# Autodesk Inventor assembly: Shoulder_nema24_v2
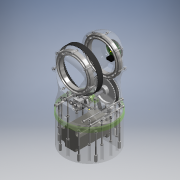
[picture p0: Inventor's stored thumbnail of the model, 180x180]
Saved by Autodesk Inventor 2016 (Build 200138000, 138)
## iProperties
Created: 2015-01-06
Part Number: Shoulder_nema24_v2
Document SubType Name: Assembly
Designer: 4ndreas
Mass: 6208.8 g
Surface Area: 5974.67 cm^2
Volume: 2503.18 cm^3
Density: 2.48036 g/cm^3
Author: 4ndreas
## Documents named in this file (30)
- C:\Users\4ndreas\Documents\Inventor\RobotARM v2\v4\Shoulder_nema24_v2.iam
- C:\Users\4ndreas\Documents\Inventor\RobotARM v2\v2\BaseJoint\Konstruktions-Assistent\Übertragung des Zahnriemens1.iam
- C:\Users\4ndreas\Documents\Inventor\Content Center Files\R2014\de-DE\DIN 125-1  A\DIN 125 - A 4,3.ipt
- C:\Users\4ndreas\Documents\Inventor\Content Center Files\R2014\de-DE\DIN BEARING(1)\DIN 625 SKF - SKF 624.ipt
- C:\Users\4ndreas\Documents\Inventor\Content Center Files\R2014\de-DE\DIN 934\DIN 934 - M4 x 0,7.ipt
- C:\Users\4ndreas\Documents\Inventor\RobotARM v2\v2\encoder.iam
- C:\Users\4ndreas\Documents\Inventor\Content Center Files\R2014\de-DE\DIN 912\DIN 912 - M4 x 0,7 x 35 x 20.ipt
- C:\Users\4ndreas\Documents\Inventor\RobotARM v2\v4\Shoulder_stepper\Konstruktions-Assistent\Übertragung des Zahnriemens1.iam
- C:\Users\4ndreas\Documents\Inventor\Content Center Files\R2014\de-DE\DIN BEARING(1)\DIN 625 SKF - SKF 61818.ipt
- C:\Users\4ndreas\Documents\Inventor\RobotARM v2\v4\Shoulder_basis_N24.ipt
- C:\Users\4ndreas\Documents\Inventor\RobotARM v2\v4\CoverBase.ipt
- C:\Users\4ndreas\Documents\Inventor\RobotARM v2\v4\Shoulder_nema24_v2\Konstruktions-Assistent\Welle1.iam
- C:\Users\4ndreas\Documents\Inventor\RobotARM v2\v4\Nema24_100.ipt
- C:\Users\4ndreas\Documents\Inventor\Content Center Files\R2014\de-DE\DIN BEARING(1)\DIN 625 SKF - SKF 608.ipt
- C:\Users\4ndreas\Documents\Inventor\Content Center Files\R2014\de-DE\DIN 125-1  A\DIN 125 - A 8,4.ipt
- C:\Users\4ndreas\Documents\Inventor\RobotARM v2\v4\LagerKlemme.ipt
- C:\Users\4ndreas\Documents\Inventor\RobotARM v2\v4\16221600.ipt
- C:\Users\4ndreas\Documents\Inventor\RobotARM v2\v4\Synchrone RiemenscheibeT5_z48.ipt
- C:\Users\4ndreas\Documents\Inventor\RobotARM v2\v4\Alu_Belt_tens.ipt
- C:\Users\4ndreas\Documents\Inventor\Content Center Files\R2014\de-DE\DIN 9021\DIN 9021 - 4,3.ipt
- C:\Users\4ndreas\Documents\Inventor\RobotARM v2\v4\DIN 912 - M4 x 0,7.ipt
- C:\Users\4ndreas\Documents\Inventor\Content Center Files\R2014\de-DE\DIN 912\DIN 912 - M4 x 0,7 x 20 x 18,25.ipt
- C:\Users\4ndreas\Documents\Inventor\Content Center Files\R2014\de-DE\DIN 912\DIN 912 - M4 x 0,7 x 25 x 23,25.ipt
- C:\Users\4ndreas\Documents\Inventor\RobotARM v2\v4\DIN 912 - M4 x 0,7 x 70.ipt
- C:\Users\4ndreas\Documents\Inventor\RobotARM v2\Diszanzbolzen_M4x20.ipt
- C:\Users\4ndreas\Documents\Inventor\Content Center Files\R2014\de-DE\DIN 562\DIN 562 - M4 x 7.ipt
- C:\Users\4ndreas\Documents\Inventor\Content Center Files\R2014\de-DE\DIN 912\DIN 912 - M4 x 0,7 x 30 x 20.ipt
- C:\Users\4ndreas\Documents\Inventor\RobotARM v2\v4\DIN 912 - M4 x 0,7 x 60.ipt
- C:\Users\4ndreas\Documents\Inventor\Content Center Files\R2014\de-DE\DIN 7991(2)\DIN 7991 - M3x25.ipt
- C:\Users\4ndreas\Documents\Inventor\Content Center Files\R2014\de-DE\DIN 934\DIN 934 - M3 x 0,5.ipt
## Components (141 placed, 28 different names)
1. Übertragung des Zahnriemens:1 [sub-assembly] — Passend:1, Passend:12, Passend:49, Passend:138, Fluchtend:18, Passend:147, Passend:173, Passend:195, Passend:228, Passend:229
2. DIN 912 - ersetzt durch DIN EN ISO 4762 M4 x 50:1 — Passend:69, Passend:82, Passend:99, Passend:179, Passend:198, Passend:203, Passend:209, Passend:210
3. DIN 625 SKF SKF 624:1 — Passend:178, Passend:192
4. DIN 625 SKF SKF 624:2 — Passend:177, Passend:186, Passend:188
5. DIN 625 SKF SKF 624:3 — Passend:80, Passend:82, Passend:181
6. DIN 625 SKF SKF 624:4 — Passend:80, Passend:180, Passend:212
7. DIN 125-1 A A 4,3:3 — Passend:193, Passend:219
8. DIN 125-1 A A 4,3:4 — Passend:183
9. DIN 125-1 A A 4,3:6 — Passend:189, Passend:194
10. DIN 934 - ersetzt durch DIN EN 24032/28673/28674 M4:1 — Passend:99, Passend:183
11. encoder:2 [sub-assembly] — Passend:116, Passend:162, Passend:163
12. Übertragung des Zahnriemens:2 [sub-assembly] — Passend:130, Passend:182
13. Nema24_100:1 — Passend:130, Winkel:10, Passend:174, Passend:175, Passend:255
14. DIN 625 SKF SKF 61818:1 — Passend:138, Passend:142, Tangential:2
15. Shoulder_basis_N24:1 — Passend:139, Fluchtend:14, Passend:140, Fluchtend:16, Passend:142, Passend:143, Passend:144, Fluchtend:17, Passend:162, Passend:163, Passend:164, Passend:169, Fluchtend:19, Passend:182, Passend:69, Passend:191, Fluchtend:20, Passend:204, Passend:205, Passend:206, Passend:208, Passend:213, Passend:221, Passend:224, Passend:225, Passend:226, Passend:227, Passend:230, Passend:293, Passend:294, Passend:295, Passend:296, Passend:297, Passend:298, Passend:299, Passend:300, Passend:301, Passend:302, Passend:303, Passend:304, Passend:305, Passend:306, Passend:307, Passend:308, Passend:309, Passend:310, Passend:311, Passend:328, Passend:329, Passend:330, Passend:331, Passend:332, Passend:333, Passend:334, Passend:335, Passend:336, Passend:337, Passend:338, Passend:339, Passend:340, Passend:341, Passend:342, Passend:344, Passend:345, Passend:346, Passend:353, Passend:354, Passend:355, Passend:356, Passend:357, Passend:358, Passend:359, Passend:367, Passend:369, Passend:370, Passend:371, Passend:374, Passend:375
16. CoverBase:1 — Passend:143, Passend:164, Passend:230, Passend:231, Passend:232, Passend:233, Passend:234, Passend:239, Passend:240, Passend:241, Passend:242, Passend:247, Passend:248, Passend:249, Passend:250, Passend:255, Passend:256, Passend:257, Passend:258, Passend:259, Passend:260, Passend:261, Passend:262, Passend:263, Passend:264, Passend:265, Passend:266, Passend:267, Passend:268, Passend:269, Passend:271, Passend:272, Passend:273, Passend:274, Passend:275, Passend:276, Passend:277, Passend:278, Passend:279, Passend:280, Passend:281, Passend:282, Passend:283, Passend:284, Passend:285, Fluchtend:31, Fluchtend:32, Passend:286, Fluchtend:33, Fluchtend:34, Fluchtend:35, Fluchtend:36, Fluchtend:37
17. DIN 625 SKF SKF 61818:2 — Passend:144, Fluchtend:17, Tangential:1
18. Welle:1 [sub-assembly] — Fluchtend:18, Passend:147, Passend:153, Passend:154, Passend:155, Passend:165, Passend:166
19. DIN 625 SKF SKF 608:1 — Passend:153, Passend:167, Passend:169
20. DIN 625 SKF SKF 608:3 — Passend:154, Passend:170, Passend:171
21. DIN 625 SKF SKF 608:4 — Passend:155
22. Synchrone RiemenscheibeT5_z48:1 — Passend:165, Passend:172
23. DIN 125-1 A A 8,4:1 — Passend:166, Passend:167, Passend:172
24. DIN 125-1 A A 8,4:2 — Passend:170, Passend:171, Passend:173
25. LagerKlemme:1 — Fluchtend:19, Passend:226, Passend:227, Passend:324, Passend:325, Passend:326, Passend:327
26. 16221600:1 — Passend:174, Passend:175
27. DIN 625 SKF SKF 624:5 — Passend:177, Passend:178, Passend:190
28. DIN 625 SKF SKF 624:6 — Passend:179, Passend:180, Passend:181
29. Alu_Belt_tens:1 — Passend:186, Passend:191, Passend:196, Passend:197, Fluchtend:20, Passend:222
30. DIN 912 - ersetzt durch DIN EN ISO 4762 M4 x 20:1 — Passend:197, Passend:200, Passend:201
31. DIN 912 - ersetzt durch DIN EN ISO 4762 M4 x 20:2 — Passend:196, Passend:199, Passend:202
32. DIN 912 - ersetzt durch DIN EN ISO 4762 M4 x 35:5 — Passend:188, Passend:189, Passend:190, Passend:192, Passend:193, Passend:194, Passend:195, Passend:207, Passend:218
33. DIN 9021 4,3:1 — Passend:198, Passend:203, Passend:204
34. DIN 9021 4,3:2 — Passend:200, Passend:201, Passend:205
35. DIN 9021 4,3:3 — Passend:199, Passend:202, Passend:206
36. DIN 9021 4,3:4 — Passend:207, Passend:208, Passend:220
37. DIN 9021 4,3:5 — Passend:209, Passend:211, Passend:213
38. DIN 934 - ersetzt durch DIN EN 24032/28673/28674 M4:2 — Passend:210, Passend:211, Passend:212
39. DIN 125-1 A A 4,3:7 — Passend:215, Passend:217, Passend:220
40. DIN 125-1 A A 4,3:8 — Passend:214, Passend:215, Passend:216
41. DIN 125-1 A A 4,3:9 — Passend:214, Passend:216, Passend:217, Passend:218, Passend:219
42. DIN 912 - ersetzt durch DIN EN ISO 4762 M4 x 25:1 — Passend:221, Passend:222, Passend:223
43. DIN 934 - ersetzt durch DIN EN 24032/28673/28674 M4:3 — Passend:223, Passend:224, Passend:225
44. DIN 912 - ersetzt durch DIN EN ISO 4762 M4 x 25:2 — Passend:233, Passend:235, Passend:245
45. DIN 912 - ersetzt durch DIN EN ISO 4762 M4 x 25:3 — Passend:232, Passend:237, Passend:243
46. DIN 912 - ersetzt durch DIN EN ISO 4762 M4 x 25:4 — Passend:231, Passend:236, Passend:244
47. DIN 912 - ersetzt durch DIN EN ISO 4762 M4 x 25:5 — Passend:234, Passend:238, Passend:246
48. DIN 125-1 A A 4,3:10 — Passend:238, Passend:239, Passend:246
49. DIN 125-1 A A 4,3:11 — Passend:237, Passend:241, Passend:243
50. DIN 125-1 A A 4,3:12 — Passend:235, Passend:242, Passend:245
51. DIN 125-1 A A 4,3:13 — Passend:236, Passend:240, Passend:244
52. DIN 625 SKF SKF 624:7 — Passend:248, Passend:251, Passend:252
53. DIN 625 SKF SKF 624:8 — Passend:247, Passend:251, Passend:253, Passend:254
54. DIN 125-1 A A 4,3:14 — Passend:249, Passend:250, Passend:252
55. DIN 125-1 A A 4,3:15 — Passend:253, Passend:254
56. DIN 912 - ersetzt durch DIN EN ISO 4762 M4 x 70:1 — Passend:259, Fluchtend:24, Fluchtend:25, Passend:291
57. DIN 912 - ersetzt durch DIN EN ISO 4762 M4 x 70:2 — Passend:263, Fluchtend:29, Passend:314
58. DIN 912 - ersetzt durch DIN EN ISO 4762 M4 x 70:3 — Passend:262, Fluchtend:29, Fluchtend:30, Passend:313
59. DIN 912 - ersetzt durch DIN EN ISO 4762 M4 x 70:4 — Passend:261, Fluchtend:28, Fluchtend:30, Passend:312
60. DIN 912 - ersetzt durch DIN EN ISO 4762 M4 x 70:5 — Passend:260, Fluchtend:25, Passend:292
61. DIN 912 - ersetzt durch DIN EN ISO 4762 M4 x 70:6 — Passend:258, Fluchtend:26, Fluchtend:27, Passend:316
62. DIN 912 - ersetzt durch DIN EN ISO 4762 M4 x 70:7 — Passend:257, Fluchtend:27, Fluchtend:28, Passend:317
63. DIN 912 - ersetzt durch DIN EN ISO 4762 M4 x 70:8 — Passend:256, Fluchtend:23, Fluchtend:24, Passend:290
64. DIN 912 - ersetzt durch DIN EN ISO 4762 M4 x 70:11 — Passend:267, Fluchtend:21, Passend:287
65. DIN 912 - ersetzt durch DIN EN ISO 4762 M4 x 70:12 — Passend:266, Fluchtend:21, Fluchtend:22, Passend:288
66. DIN 912 - ersetzt durch DIN EN ISO 4762 M4 x 70:13 — Passend:265, Fluchtend:22, Fluchtend:23, Passend:289
67. DIN 912 - ersetzt durch DIN EN ISO 4762 M4 x 70:14 — Passend:264, Fluchtend:26, Passend:315
68. DIN 912 - ersetzt durch DIN EN ISO 4762 M4 x 70:15 — Passend:268, Passend:269, Passend:270, Fluchtend:45, Fluchtend:46
69. Diszanzbolzen_M4x20:1 — Passend:270, Passend:278, Passend:279
70. Diszanzbolzen_M4x20:2 — Passend:271, Passend:283, Fluchtend:36, Passend:366
71. Diszanzbolzen_M4x20:3 — Passend:272, Passend:284, Fluchtend:37, Passend:365
72. Diszanzbolzen_M4x20:4 — Passend:276, Passend:281, Fluchtend:34, Passend:361
73. Diszanzbolzen_M4x20:5 — Passend:275, Passend:280, Fluchtend:33, Passend:362
74. Diszanzbolzen_M4x20:6 — Passend:274, Fluchtend:32, Passend:286, Passend:363
75. Diszanzbolzen_M4x20:7 — Passend:273, Passend:285, Fluchtend:31, Passend:364
76. Diszanzbolzen_M4x20:8 — Passend:277, Passend:282, Fluchtend:35, Passend:360
77. DIN 934 - ersetzt durch DIN EN 24032/28673/28674 M4:4 — Passend:287, Fluchtend:42, Passend:293
78. DIN 934 - ersetzt durch DIN EN 24032/28673/28674 M4:5 — Passend:288, Fluchtend:40, Fluchtend:41, Passend:294
79. DIN 934 - ersetzt durch DIN EN 24032/28673/28674 M4:6 — Passend:289, Fluchtend:41, Fluchtend:42, Passend:295
80. DIN 934 - ersetzt durch DIN EN 24032/28673/28674 M4:7 — Passend:290, Fluchtend:38, Passend:296
81. DIN 934 - ersetzt durch DIN EN 24032/28673/28674 M4:10 — Passend:292, Fluchtend:39, Fluchtend:40, Passend:298
82. DIN 934 - ersetzt durch DIN EN 24032/28673/28674 M4:11 — Passend:291, Fluchtend:38, Fluchtend:39, Passend:297, Passend:299
83. DIN 562 M4:1 — Passend:300, Passend:301, Passend:317
84. DIN 562 M4:2 — Passend:302, Passend:303, Passend:316
85. DIN 562 M4:3 — Passend:304, Passend:305, Passend:315
86. DIN 562 M4:4 — Passend:307, Passend:310, Passend:313
87. DIN 562 M4:5 — Passend:306, Passend:311, Passend:312
88. DIN 562 M4:6 — Passend:308, Passend:309, Passend:314
89. DIN 912 - ersetzt durch DIN EN ISO 4762 M4 x 30:1 — Passend:318, Passend:321, Passend:322, Passend:324
90. DIN 912 - ersetzt durch DIN EN ISO 4762 M4 x 30:2 — Passend:319, Passend:320, Passend:323, Passend:326
91. DIN 934 - ersetzt durch DIN EN 24032/28673/28674 M4:12 — Passend:319, Fluchtend:43, Passend:329
92. DIN 934 - ersetzt durch DIN EN 24032/28673/28674 M4:13 — Passend:318, Fluchtend:43, Passend:328, Passend:330
93. DIN 125-1 A A 4,3:16 — Passend:321, Passend:322, Passend:325
94. DIN 125-1 A A 4,3:17 — Passend:320, Passend:323, Passend:327
95. Diszanzbolzen_M4x20:9 — Passend:333, Passend:339, Passend:342, Passend:347
96. Diszanzbolzen_M4x20:10 — Passend:334, Passend:340, Passend:341, Passend:351
97. Diszanzbolzen_M4x20:11 — Passend:331, Passend:335, Passend:338, Passend:349
98. Diszanzbolzen_M4x20:12 — Passend:332, Passend:336, Passend:337
99. DIN 912 - ersetzt durch DIN EN ISO 4762 M4 x 50:2 — Passend:344, Passend:346
100. DIN 912 - ersetzt durch DIN EN ISO 4762 M4 x 50:3 — Passend:347, Passend:348, Passend:359
101. DIN 912 - ersetzt durch DIN EN ISO 4762 M4 x 50:4 — Passend:348, Passend:353
102. DIN 912 - ersetzt durch DIN EN ISO 4762 M4 x 50:5 — Passend:345, Passend:356
103. DIN 912 - ersetzt durch DIN EN ISO 4762 M4 x 60:16 — Passend:350, Passend:355
104. DIN 912 - ersetzt durch DIN EN ISO 4762 M4 x 60:17 — Passend:349, Passend:350, Passend:357
105. DIN 912 - ersetzt durch DIN EN ISO 4762 M4 x 60:18 — Passend:352, Passend:354
106. DIN 912 - ersetzt durch DIN EN ISO 4762 M4 x 60:19 — Passend:351, Passend:352, Passend:358
107. DIN 912 - ersetzt durch DIN EN ISO 4762 M4 x 70:20 — Passend:361, Fluchtend:47, Fluchtend:48, Fluchtend:49
108. DIN 912 - ersetzt durch DIN EN ISO 4762 M4 x 70:21 — Passend:362, Fluchtend:47
109. DIN 912 - ersetzt durch DIN EN ISO 4762 M4 x 70:22 — Passend:364, Fluchtend:50
110. DIN 912 - ersetzt durch DIN EN ISO 4762 M4 x 70:24 — Passend:363, Fluchtend:49, Fluchtend:50
111. DIN 912 - ersetzt durch DIN EN ISO 4762 M4 x 70:25 — Passend:360, Fluchtend:46, Fluchtend:48
112. DIN 912 - ersetzt durch DIN EN ISO 4762 M4 x 70:26 — Passend:365, Fluchtend:44
113. DIN 912 - ersetzt durch DIN EN ISO 4762 M4 x 70:27 — Passend:366, Fluchtend:44, Fluchtend:45
114. DIN 934 - ersetzt durch DIN EN 24032/28673/28674 M3:1 — Passend:368, Passend:369, Passend:370
115. DIN 7991 M3x25:1 — Passend:367, Tangential:1, Passend:368
116. DIN 934 - ersetzt durch DIN EN 24032/28673/28674 M3:2
117. DIN 7991 M3x25:2
118. DIN 934 - ersetzt durch DIN EN 24032/28673/28674 M3:3
119. DIN 7991 M3x25:3
120. DIN 934 - ersetzt durch DIN EN 24032/28673/28674 M3:4
121. DIN 7991 M3x25:4
122. DIN 934 - ersetzt durch DIN EN 24032/28673/28674 M3:5
123. DIN 7991 M3x25:5
124. DIN 934 - ersetzt durch DIN EN 24032/28673/28674 M3:6
125. DIN 7991 M3x25:6
126. DIN 934 - ersetzt durch DIN EN 24032/28673/28674 M3:7
127. DIN 7991 M3x25:7
128. DIN 7991 M3x25:8 — Passend:371, Passend:373, Tangential:2
129. DIN 934 - ersetzt durch DIN EN 24032/28673/28674 M3:8 — Passend:373, Passend:374, Passend:375
130. DIN 7991 M3x25:9
131. DIN 934 - ersetzt durch DIN EN 24032/28673/28674 M3:9
132. DIN 7991 M3x25:10
133. DIN 934 - ersetzt durch DIN EN 24032/28673/28674 M3:10
134. DIN 7991 M3x25:11
135. DIN 934 - ersetzt durch DIN EN 24032/28673/28674 M3:11
136. DIN 7991 M3x25:12
137. DIN 934 - ersetzt durch DIN EN 24032/28673/28674 M3:12
138. DIN 7991 M3x25:13
139. DIN 934 - ersetzt durch DIN EN 24032/28673/28674 M3:13
140. DIN 7991 M3x25:14
141. DIN 934 - ersetzt durch DIN EN 24032/28673/28674 M3:14
## Component patterns: (7 elements, first: DIN 934 - ersetzt durch DIN EN 24032/28673/28674 M3:1 + DIN 7991 M3x25:1), (7 elements, first: DIN 7991 M3x25:8 + DIN 934 - ersetzt durch DIN EN 24032/28673/28674 M3:8)
## Relationships (274: Mate 233, Flush 38, Tangent 2, Angle 1)
- Passend:1 [Mate]: Übertragung des Zahnriemens:1
- Passend:4 [Mate]
- Passend:12 [Mate]: Übertragung des Zahnriemens:1
- Passend:49 [Mate]: Übertragung des Zahnriemens:1
- Passend:62 [Mate]
- Passend:63 [Mate]
- Passend:69 [Mate]: DIN 912 - ersetzt durch DIN EN ISO 4762 M4 x 50:1 ↔ Shoulder_basis_N24:1
- Passend:80 [Mate]: DIN 625 SKF SKF 624:3 ↔ DIN 625 SKF SKF 624:4
- Passend:82 [Mate]: DIN 912 - ersetzt durch DIN EN ISO 4762 M4 x 50:1 ↔ DIN 625 SKF SKF 624:3
- [Mate]: DIN 912 - ersetzt durch DIN EN ISO 4762 M4 x 50:1 ↔ DIN 125-1 A A 4,3:4
- [Mate]: DIN 625 SKF SKF 624:3 ↔ DIN 125-1 A A 4,3:4
- [Mate]: DIN 625 SKF SKF 624:2 ↔ DIN 125-1 A A 4,3:6
- [Mate]: DIN 625 SKF SKF 624:1 ↔ DIN 125-1 A A 4,3:3
- Passend:99 [Mate]: DIN 912 - ersetzt durch DIN EN ISO 4762 M4 x 50:1 ↔ DIN 934 - ersetzt durch DIN EN 24032/28673/28674 M4:1
- Passend:116 [Mate]: encoder:2
- Fluchtend:12 [Flush] (43 mm)
- Fluchtend:13 [Flush] (20 mm)
- Passend:130 [Mate]: Übertragung des Zahnriemens:2 ↔ Nema24_100:1
- Winkel:10 [Angle] (0 deg): Nema24_100:1
- Passend:138 [Mate]: Übertragung des Zahnriemens:1 ↔ DIN 625 SKF SKF 61818:1
- Passend:139 [Mate]: Shoulder_basis_N24:1
- Fluchtend:14 [Flush]: Shoulder_basis_N24:1
- Passend:140 [Mate]: Shoulder_basis_N24:1
- Fluchtend:16 [Flush]: Shoulder_basis_N24:1
- Passend:142 [Mate]: DIN 625 SKF SKF 61818:1 ↔ Shoulder_basis_N24:1
- Passend:143 [Mate]: Shoulder_basis_N24:1 ↔ CoverBase:1
- Passend:144 [Mate]: Shoulder_basis_N24:1 ↔ DIN 625 SKF SKF 61818:2
- Fluchtend:17 [Flush]: Shoulder_basis_N24:1 ↔ DIN 625 SKF SKF 61818:2
- Fluchtend:18 [Flush] (-10 mm): Übertragung des Zahnriemens:1 ↔ Welle:1
- Passend:147 [Mate]: Übertragung des Zahnriemens:1 ↔ Welle:1
- Passend:153 [Mate]: Welle:1 ↔ DIN 625 SKF SKF 608:1
- Passend:154 [Mate]: Welle:1 ↔ DIN 625 SKF SKF 608:3
- Passend:155 [Mate]: Welle:1 ↔ DIN 625 SKF SKF 608:4
- Passend:162 [Mate]: encoder:2 ↔ Shoulder_basis_N24:1
- Passend:163 [Mate]: encoder:2 ↔ Shoulder_basis_N24:1
- Passend:164 [Mate]: Shoulder_basis_N24:1 ↔ CoverBase:1
- Passend:165 [Mate]: Welle:1 ↔ Synchrone RiemenscheibeT5_z48:1
- Passend:166 [Mate]: Welle:1 ↔ DIN 125-1 A A 8,4:1
- Passend:167 [Mate]: DIN 625 SKF SKF 608:1 ↔ DIN 125-1 A A 8,4:1
- Passend:169 [Mate]: Shoulder_basis_N24:1 ↔ DIN 625 SKF SKF 608:1
- Passend:170 [Mate]: DIN 625 SKF SKF 608:3 ↔ DIN 125-1 A A 8,4:2
- Passend:171 [Mate]: DIN 625 SKF SKF 608:3 ↔ DIN 125-1 A A 8,4:2
- Passend:172 [Mate]: Synchrone RiemenscheibeT5_z48:1 ↔ DIN 125-1 A A 8,4:1
- Passend:173 [Mate] (0.5 mm): Übertragung des Zahnriemens:1 ↔ DIN 125-1 A A 8,4:2
- Fluchtend:19 [Flush]: Shoulder_basis_N24:1 ↔ LagerKlemme:1
- Passend:174 [Mate]: Nema24_100:1 ↔ 16221600:1
- Passend:175 [Mate] (0.5 mm): Nema24_100:1 ↔ 16221600:1
- Passend:177 [Mate]: DIN 625 SKF SKF 624:2 ↔ DIN 625 SKF SKF 624:5
- Passend:178 [Mate]: DIN 625 SKF SKF 624:1 ↔ DIN 625 SKF SKF 624:5
- Passend:179 [Mate]: DIN 912 - ersetzt durch DIN EN ISO 4762 M4 x 50:1 ↔ DIN 625 SKF SKF 624:6
- Passend:180 [Mate]: DIN 625 SKF SKF 624:4 ↔ DIN 625 SKF SKF 624:6
- Passend:181 [Mate]: DIN 625 SKF SKF 624:3 ↔ DIN 625 SKF SKF 624:6
- Passend:182 [Mate]: Übertragung des Zahnriemens:2 ↔ Shoulder_basis_N24:1
- Passend:183 [Mate]: DIN 125-1 A A 4,3:4 ↔ DIN 934 - ersetzt durch DIN EN 24032/28673/28674 M4:1
- Passend:186 [Mate]: DIN 625 SKF SKF 624:2 ↔ Alu_Belt_tens:1
- Passend:188 [Mate]: DIN 625 SKF SKF 624:2 ↔ DIN 912 - ersetzt durch DIN EN ISO 4762 M4 x 35:5
- Passend:189 [Mate]: DIN 125-1 A A 4,3:6 ↔ DIN 912 - ersetzt durch DIN EN ISO 4762 M4 x 35:5
- Passend:190 [Mate]: DIN 625 SKF SKF 624:5 ↔ DIN 912 - ersetzt durch DIN EN ISO 4762 M4 x 35:5
- Passend:191 [Mate]: Shoulder_basis_N24:1 ↔ Alu_Belt_tens:1
- Passend:192 [Mate]: DIN 625 SKF SKF 624:1 ↔ DIN 912 - ersetzt durch DIN EN ISO 4762 M4 x 35:5
- Passend:193 [Mate]: DIN 125-1 A A 4,3:3 ↔ DIN 912 - ersetzt durch DIN EN ISO 4762 M4 x 35:5
- Passend:194 [Mate]: DIN 125-1 A A 4,3:6 ↔ DIN 912 - ersetzt durch DIN EN ISO 4762 M4 x 35:5
- Passend:195 [Mate]: Übertragung des Zahnriemens:1 ↔ DIN 912 - ersetzt durch DIN EN ISO 4762 M4 x 35:5
- Passend:196 [Mate]: Alu_Belt_tens:1 ↔ DIN 912 - ersetzt durch DIN EN ISO 4762 M4 x 20:2
- Passend:197 [Mate]: Alu_Belt_tens:1 ↔ DIN 912 - ersetzt durch DIN EN ISO 4762 M4 x 20:1
- Fluchtend:20 [Flush]: Shoulder_basis_N24:1 ↔ Alu_Belt_tens:1
- Passend:198 [Mate]: DIN 912 - ersetzt durch DIN EN ISO 4762 M4 x 50:1 ↔ DIN 9021 4,3:1
- Passend:199 [Mate]: DIN 912 - ersetzt durch DIN EN ISO 4762 M4 x 20:2 ↔ DIN 9021 4,3:3
- Passend:200 [Mate]: DIN 912 - ersetzt durch DIN EN ISO 4762 M4 x 20:1 ↔ DIN 9021 4,3:2
- Passend:201 [Mate]: DIN 912 - ersetzt durch DIN EN ISO 4762 M4 x 20:1 ↔ DIN 9021 4,3:2
- Passend:202 [Mate]: DIN 912 - ersetzt durch DIN EN ISO 4762 M4 x 20:2 ↔ DIN 9021 4,3:3
- Passend:203 [Mate]: DIN 912 - ersetzt durch DIN EN ISO 4762 M4 x 50:1 ↔ DIN 9021 4,3:1
- Passend:204 [Mate]: Shoulder_basis_N24:1 ↔ DIN 9021 4,3:1
- Passend:205 [Mate]: Shoulder_basis_N24:1 ↔ DIN 9021 4,3:2
- Passend:206 [Mate]: Shoulder_basis_N24:1 ↔ DIN 9021 4,3:3
- Passend:207 [Mate]: DIN 912 - ersetzt durch DIN EN ISO 4762 M4 x 35:5 ↔ DIN 9021 4,3:4
- Passend:208 [Mate]: Shoulder_basis_N24:1 ↔ DIN 9021 4,3:4
- Passend:209 [Mate]: DIN 912 - ersetzt durch DIN EN ISO 4762 M4 x 50:1 ↔ DIN 9021 4,3:5
- Passend:210 [Mate]: DIN 912 - ersetzt durch DIN EN ISO 4762 M4 x 50:1 ↔ DIN 934 - ersetzt durch DIN EN 24032/28673/28674 M4:2
- Passend:211 [Mate]: DIN 9021 4,3:5 ↔ DIN 934 - ersetzt durch DIN EN 24032/28673/28674 M4:2
- Passend:212 [Mate]: DIN 625 SKF SKF 624:4 ↔ DIN 934 - ersetzt durch DIN EN 24032/28673/28674 M4:2
- Passend:213 [Mate]: Shoulder_basis_N24:1 ↔ DIN 9021 4,3:5
- Passend:214 [Mate]: DIN 125-1 A A 4,3:8 ↔ DIN 125-1 A A 4,3:9
- Passend:215 [Mate]: DIN 125-1 A A 4,3:7 ↔ DIN 125-1 A A 4,3:8
- Passend:216 [Mate]: DIN 125-1 A A 4,3:8 ↔ DIN 125-1 A A 4,3:9
- Passend:217 [Mate]: DIN 125-1 A A 4,3:7 ↔ DIN 125-1 A A 4,3:9
- Passend:218 [Mate]: DIN 912 - ersetzt durch DIN EN ISO 4762 M4 x 35:5 ↔ DIN 125-1 A A 4,3:9
- Passend:219 [Mate]: DIN 125-1 A A 4,3:3 ↔ DIN 125-1 A A 4,3:9
- Passend:220 [Mate]: DIN 9021 4,3:4 ↔ DIN 125-1 A A 4,3:7
- Passend:221 [Mate]: Shoulder_basis_N24:1 ↔ DIN 912 - ersetzt durch DIN EN ISO 4762 M4 x 25:1
- Passend:222 [Mate]: Alu_Belt_tens:1 ↔ DIN 912 - ersetzt durch DIN EN ISO 4762 M4 x 25:1
- Passend:223 [Mate]: DIN 912 - ersetzt durch DIN EN ISO 4762 M4 x 25:1 ↔ DIN 934 - ersetzt durch DIN EN 24032/28673/28674 M4:3
- Passend:224 [Mate]: Shoulder_basis_N24:1 ↔ DIN 934 - ersetzt durch DIN EN 24032/28673/28674 M4:3
- Passend:225 [Mate]: Shoulder_basis_N24:1 ↔ DIN 934 - ersetzt durch DIN EN 24032/28673/28674 M4:3
- Passend:226 [Mate]: Shoulder_basis_N24:1 ↔ LagerKlemme:1
- Passend:227 [Mate]: Shoulder_basis_N24:1 ↔ LagerKlemme:1
- Passend:228 [Mate]: Übertragung des Zahnriemens:1
- Passend:229 [Mate]: Übertragung des Zahnriemens:1
- Passend:230 [Mate]: Shoulder_basis_N24:1 ↔ CoverBase:1
- Passend:231 [Mate]: CoverBase:1 ↔ DIN 912 - ersetzt durch DIN EN ISO 4762 M4 x 25:4
- Passend:232 [Mate]: CoverBase:1 ↔ DIN 912 - ersetzt durch DIN EN ISO 4762 M4 x 25:3
- Passend:233 [Mate]: CoverBase:1 ↔ DIN 912 - ersetzt durch DIN EN ISO 4762 M4 x 25:2
- Passend:234 [Mate]: CoverBase:1 ↔ DIN 912 - ersetzt durch DIN EN ISO 4762 M4 x 25:5
- Passend:235 [Mate]: DIN 912 - ersetzt durch DIN EN ISO 4762 M4 x 25:2 ↔ DIN 125-1 A A 4,3:12
- Passend:236 [Mate]: DIN 912 - ersetzt durch DIN EN ISO 4762 M4 x 25:4 ↔ DIN 125-1 A A 4,3:13
- Passend:237 [Mate]: DIN 912 - ersetzt durch DIN EN ISO 4762 M4 x 25:3 ↔ DIN 125-1 A A 4,3:11
- Passend:238 [Mate]: DIN 912 - ersetzt durch DIN EN ISO 4762 M4 x 25:5 ↔ DIN 125-1 A A 4,3:10
- Passend:239 [Mate]: CoverBase:1 ↔ DIN 125-1 A A 4,3:10
- Passend:240 [Mate]: CoverBase:1 ↔ DIN 125-1 A A 4,3:13
- Passend:241 [Mate]: CoverBase:1 ↔ DIN 125-1 A A 4,3:11
- Passend:242 [Mate]: CoverBase:1 ↔ DIN 125-1 A A 4,3:12
- Passend:243 [Mate]: DIN 912 - ersetzt durch DIN EN ISO 4762 M4 x 25:3 ↔ DIN 125-1 A A 4,3:11
- Passend:244 [Mate]: DIN 912 - ersetzt durch DIN EN ISO 4762 M4 x 25:4 ↔ DIN 125-1 A A 4,3:13
- Passend:245 [Mate]: DIN 912 - ersetzt durch DIN EN ISO 4762 M4 x 25:2 ↔ DIN 125-1 A A 4,3:12
- Passend:246 [Mate]: DIN 912 - ersetzt durch DIN EN ISO 4762 M4 x 25:5 ↔ DIN 125-1 A A 4,3:10
- Passend:247 [Mate]: CoverBase:1 ↔ DIN 625 SKF SKF 624:8
- Passend:248 [Mate]: CoverBase:1 ↔ DIN 625 SKF SKF 624:7
- Passend:249 [Mate]: CoverBase:1 ↔ DIN 125-1 A A 4,3:14
- Passend:250 [Mate]: CoverBase:1 ↔ DIN 125-1 A A 4,3:14
- Passend:251 [Mate]: DIN 625 SKF SKF 624:7 ↔ DIN 625 SKF SKF 624:8
- Passend:252 [Mate]: DIN 625 SKF SKF 624:7 ↔ DIN 125-1 A A 4,3:14
- Passend:253 [Mate]: DIN 625 SKF SKF 624:8 ↔ DIN 125-1 A A 4,3:15
- Passend:254 [Mate]: DIN 625 SKF SKF 624:8 ↔ DIN 125-1 A A 4,3:15
- Passend:255 [Mate]: Nema24_100:1 ↔ CoverBase:1
- Passend:256 [Mate]: CoverBase:1 ↔ DIN 912 - ersetzt durch DIN EN ISO 4762 M4 x 70:8
- Passend:257 [Mate]: CoverBase:1 ↔ DIN 912 - ersetzt durch DIN EN ISO 4762 M4 x 70:7
- Passend:258 [Mate]: CoverBase:1 ↔ DIN 912 - ersetzt durch DIN EN ISO 4762 M4 x 70:6
- Passend:259 [Mate]: CoverBase:1 ↔ DIN 912 - ersetzt durch DIN EN ISO 4762 M4 x 70:1
- Passend:260 [Mate]: CoverBase:1 ↔ DIN 912 - ersetzt durch DIN EN ISO 4762 M4 x 70:5
- Passend:261 [Mate]: CoverBase:1 ↔ DIN 912 - ersetzt durch DIN EN ISO 4762 M4 x 70:4
- Passend:262 [Mate]: CoverBase:1 ↔ DIN 912 - ersetzt durch DIN EN ISO 4762 M4 x 70:3
- Passend:263 [Mate]: CoverBase:1 ↔ DIN 912 - ersetzt durch DIN EN ISO 4762 M4 x 70:2
- Passend:264 [Mate]: CoverBase:1 ↔ DIN 912 - ersetzt durch DIN EN ISO 4762 M4 x 70:14
- Passend:265 [Mate]: CoverBase:1 ↔ DIN 912 - ersetzt durch DIN EN ISO 4762 M4 x 70:13
- Passend:266 [Mate]: CoverBase:1 ↔ DIN 912 - ersetzt durch DIN EN ISO 4762 M4 x 70:12
- Passend:267 [Mate]: CoverBase:1 ↔ DIN 912 - ersetzt durch DIN EN ISO 4762 M4 x 70:11
- Fluchtend:21 [Flush]: DIN 912 - ersetzt durch DIN EN ISO 4762 M4 x 70:11 ↔ DIN 912 - ersetzt durch DIN EN ISO 4762 M4 x 70:12
- Fluchtend:22 [Flush]: DIN 912 - ersetzt durch DIN EN ISO 4762 M4 x 70:12 ↔ DIN 912 - ersetzt durch DIN EN ISO 4762 M4 x 70:13
- Fluchtend:23 [Flush]: DIN 912 - ersetzt durch DIN EN ISO 4762 M4 x 70:8 ↔ DIN 912 - ersetzt durch DIN EN ISO 4762 M4 x 70:13
- Fluchtend:24 [Flush]: DIN 912 - ersetzt durch DIN EN ISO 4762 M4 x 70:1 ↔ DIN 912 - ersetzt durch DIN EN ISO 4762 M4 x 70:8
- Fluchtend:25 [Flush]: DIN 912 - ersetzt durch DIN EN ISO 4762 M4 x 70:1 ↔ DIN 912 - ersetzt durch DIN EN ISO 4762 M4 x 70:5
- Fluchtend:26 [Flush]: DIN 912 - ersetzt durch DIN EN ISO 4762 M4 x 70:6 ↔ DIN 912 - ersetzt durch DIN EN ISO 4762 M4 x 70:14
- Fluchtend:27 [Flush]: DIN 912 - ersetzt durch DIN EN ISO 4762 M4 x 70:6 ↔ DIN 912 - ersetzt durch DIN EN ISO 4762 M4 x 70:7
- Fluchtend:28 [Flush]: DIN 912 - ersetzt durch DIN EN ISO 4762 M4 x 70:4 ↔ DIN 912 - ersetzt durch DIN EN ISO 4762 M4 x 70:7
- Fluchtend:29 [Flush]: DIN 912 - ersetzt durch DIN EN ISO 4762 M4 x 70:2 ↔ DIN 912 - ersetzt durch DIN EN ISO 4762 M4 x 70:3
- Fluchtend:30 [Flush]: DIN 912 - ersetzt durch DIN EN ISO 4762 M4 x 70:3 ↔ DIN 912 - ersetzt durch DIN EN ISO 4762 M4 x 70:4
- Passend:268 [Mate]: CoverBase:1 ↔ DIN 912 - ersetzt durch DIN EN ISO 4762 M4 x 70:15
- Passend:269 [Mate]: CoverBase:1 ↔ DIN 912 - ersetzt durch DIN EN ISO 4762 M4 x 70:15
- Passend:270 [Mate]: DIN 912 - ersetzt durch DIN EN ISO 4762 M4 x 70:15 ↔ Diszanzbolzen_M4x20:1
- Passend:271 [Mate]: CoverBase:1 ↔ Diszanzbolzen_M4x20:2
- Passend:272 [Mate]: CoverBase:1 ↔ Diszanzbolzen_M4x20:3
- Passend:273 [Mate]: CoverBase:1 ↔ Diszanzbolzen_M4x20:7
- Passend:274 [Mate]: CoverBase:1 ↔ Diszanzbolzen_M4x20:6
- Passend:275 [Mate]: CoverBase:1 ↔ Diszanzbolzen_M4x20:5
- Passend:276 [Mate]: CoverBase:1 ↔ Diszanzbolzen_M4x20:4
- Passend:277 [Mate]: CoverBase:1 ↔ Diszanzbolzen_M4x20:8
- Passend:278 [Mate]: CoverBase:1 ↔ Diszanzbolzen_M4x20:1
- Passend:279 [Mate]: CoverBase:1 ↔ Diszanzbolzen_M4x20:1
- Passend:280 [Mate]: CoverBase:1 ↔ Diszanzbolzen_M4x20:5
- Passend:281 [Mate]: CoverBase:1 ↔ Diszanzbolzen_M4x20:4
- Passend:282 [Mate]: CoverBase:1 ↔ Diszanzbolzen_M4x20:8
- Passend:283 [Mate]: CoverBase:1 ↔ Diszanzbolzen_M4x20:2
- Passend:284 [Mate]: CoverBase:1 ↔ Diszanzbolzen_M4x20:3
- Passend:285 [Mate]: CoverBase:1 ↔ Diszanzbolzen_M4x20:7
- Fluchtend:31 [Flush]: CoverBase:1 ↔ Diszanzbolzen_M4x20:7
- Fluchtend:32 [Flush]: CoverBase:1 ↔ Diszanzbolzen_M4x20:6
- Passend:286 [Mate]: CoverBase:1 ↔ Diszanzbolzen_M4x20:6
- Fluchtend:33 [Flush]: CoverBase:1 ↔ Diszanzbolzen_M4x20:5
- Fluchtend:34 [Flush]: CoverBase:1 ↔ Diszanzbolzen_M4x20:4
- Fluchtend:35 [Flush]: CoverBase:1 ↔ Diszanzbolzen_M4x20:8
- Fluchtend:36 [Flush]: CoverBase:1 ↔ Diszanzbolzen_M4x20:2
- Fluchtend:37 [Flush]: CoverBase:1 ↔ Diszanzbolzen_M4x20:3
- Passend:287 [Mate]: DIN 912 - ersetzt durch DIN EN ISO 4762 M4 x 70:11 ↔ DIN 934 - ersetzt durch DIN EN 24032/28673/28674 M4:4
- Passend:288 [Mate]: DIN 912 - ersetzt durch DIN EN ISO 4762 M4 x 70:12 ↔ DIN 934 - ersetzt durch DIN EN 24032/28673/28674 M4:5
- Passend:289 [Mate]: DIN 912 - ersetzt durch DIN EN ISO 4762 M4 x 70:13 ↔ DIN 934 - ersetzt durch DIN EN 24032/28673/28674 M4:6
- Passend:290 [Mate]: DIN 912 - ersetzt durch DIN EN ISO 4762 M4 x 70:8 ↔ DIN 934 - ersetzt durch DIN EN 24032/28673/28674 M4:7
- Passend:291 [Mate]: DIN 912 - ersetzt durch DIN EN ISO 4762 M4 x 70:1 ↔ DIN 934 - ersetzt durch DIN EN 24032/28673/28674 M4:11
- Passend:292 [Mate]: DIN 912 - ersetzt durch DIN EN ISO 4762 M4 x 70:5 ↔ DIN 934 - ersetzt durch DIN EN 24032/28673/28674 M4:10
- Fluchtend:38 [Flush]: DIN 934 - ersetzt durch DIN EN 24032/28673/28674 M4:7 ↔ DIN 934 - ersetzt durch DIN EN 24032/28673/28674 M4:11
- Fluchtend:39 [Flush]: DIN 934 - ersetzt durch DIN EN 24032/28673/28674 M4:10 ↔ DIN 934 - ersetzt durch DIN EN 24032/28673/28674 M4:11
- Fluchtend:40 [Flush]: DIN 934 - ersetzt durch DIN EN 24032/28673/28674 M4:5 ↔ DIN 934 - ersetzt durch DIN EN 24032/28673/28674 M4:10
- Fluchtend:41 [Flush]: DIN 934 - ersetzt durch DIN EN 24032/28673/28674 M4:5 ↔ DIN 934 - ersetzt durch DIN EN 24032/28673/28674 M4:6
- Fluchtend:42 [Flush]: DIN 934 - ersetzt durch DIN EN 24032/28673/28674 M4:4 ↔ DIN 934 - ersetzt durch DIN EN 24032/28673/28674 M4:6
- Passend:293 [Mate]: Shoulder_basis_N24:1 ↔ DIN 934 - ersetzt durch DIN EN 24032/28673/28674 M4:4
- Passend:294 [Mate]: Shoulder_basis_N24:1 ↔ DIN 934 - ersetzt durch DIN EN 24032/28673/28674 M4:5
- Passend:295 [Mate]: Shoulder_basis_N24:1 ↔ DIN 934 - ersetzt durch DIN EN 24032/28673/28674 M4:6
- Passend:296 [Mate]: Shoulder_basis_N24:1 ↔ DIN 934 - ersetzt durch DIN EN 24032/28673/28674 M4:7
- Passend:297 [Mate]: Shoulder_basis_N24:1 ↔ DIN 934 - ersetzt durch DIN EN 24032/28673/28674 M4:11
- Passend:298 [Mate]: Shoulder_basis_N24:1 ↔ DIN 934 - ersetzt durch DIN EN 24032/28673/28674 M4:10
- Passend:299 [Mate]: Shoulder_basis_N24:1 ↔ DIN 934 - ersetzt durch DIN EN 24032/28673/28674 M4:11
- Passend:300 [Mate]: Shoulder_basis_N24:1 ↔ DIN 562 M4:1
- Passend:301 [Mate]: Shoulder_basis_N24:1 ↔ DIN 562 M4:1
- Passend:302 [Mate]: Shoulder_basis_N24:1 ↔ DIN 562 M4:2
- Passend:303 [Mate]: Shoulder_basis_N24:1 ↔ DIN 562 M4:2
- Passend:304 [Mate]: Shoulder_basis_N24:1 ↔ DIN 562 M4:3
- Passend:305 [Mate]: Shoulder_basis_N24:1 ↔ DIN 562 M4:3
- Passend:306 [Mate]: Shoulder_basis_N24:1 ↔ DIN 562 M4:5
- Passend:307 [Mate]: Shoulder_basis_N24:1 ↔ DIN 562 M4:4
- Passend:308 [Mate]: Shoulder_basis_N24:1 ↔ DIN 562 M4:6
- Passend:309 [Mate]: Shoulder_basis_N24:1 ↔ DIN 562 M4:6
- Passend:310 [Mate]: Shoulder_basis_N24:1 ↔ DIN 562 M4:4
- Passend:311 [Mate]: Shoulder_basis_N24:1 ↔ DIN 562 M4:5
- Passend:312 [Mate]: DIN 912 - ersetzt durch DIN EN ISO 4762 M4 x 70:4 ↔ DIN 562 M4:5
- Passend:313 [Mate]: DIN 912 - ersetzt durch DIN EN ISO 4762 M4 x 70:3 ↔ DIN 562 M4:4
- Passend:314 [Mate]: DIN 912 - ersetzt durch DIN EN ISO 4762 M4 x 70:2 ↔ DIN 562 M4:6
- Passend:315 [Mate]: DIN 912 - ersetzt durch DIN EN ISO 4762 M4 x 70:14 ↔ DIN 562 M4:3
- Passend:316 [Mate]: DIN 912 - ersetzt durch DIN EN ISO 4762 M4 x 70:6 ↔ DIN 562 M4:2
- Passend:317 [Mate]: DIN 912 - ersetzt durch DIN EN ISO 4762 M4 x 70:7 ↔ DIN 562 M4:1
- Passend:318 [Mate]: DIN 912 - ersetzt durch DIN EN ISO 4762 M4 x 30:1 ↔ DIN 934 - ersetzt durch DIN EN 24032/28673/28674 M4:13
- Passend:319 [Mate]: DIN 912 - ersetzt durch DIN EN ISO 4762 M4 x 30:2 ↔ DIN 934 - ersetzt durch DIN EN 24032/28673/28674 M4:12
- Passend:320 [Mate]: DIN 912 - ersetzt durch DIN EN ISO 4762 M4 x 30:2 ↔ DIN 125-1 A A 4,3:17
- Passend:321 [Mate]: DIN 912 - ersetzt durch DIN EN ISO 4762 M4 x 30:1 ↔ DIN 125-1 A A 4,3:16
- Passend:322 [Mate]: DIN 912 - ersetzt durch DIN EN ISO 4762 M4 x 30:1 ↔ DIN 125-1 A A 4,3:16
- Passend:323 [Mate]: DIN 912 - ersetzt durch DIN EN ISO 4762 M4 x 30:2 ↔ DIN 125-1 A A 4,3:17
- Passend:324 [Mate]: LagerKlemme:1 ↔ DIN 912 - ersetzt durch DIN EN ISO 4762 M4 x 30:1
- Passend:325 [Mate]: LagerKlemme:1 ↔ DIN 125-1 A A 4,3:16
- Passend:326 [Mate]: LagerKlemme:1 ↔ DIN 912 - ersetzt durch DIN EN ISO 4762 M4 x 30:2
- Passend:327 [Mate]: LagerKlemme:1 ↔ DIN 125-1 A A 4,3:17
- Fluchtend:43 [Flush]: DIN 934 - ersetzt durch DIN EN 24032/28673/28674 M4:12 ↔ DIN 934 - ersetzt durch DIN EN 24032/28673/28674 M4:13
- Passend:328 [Mate]: Shoulder_basis_N24:1 ↔ DIN 934 - ersetzt durch DIN EN 24032/28673/28674 M4:13
- Passend:329 [Mate]: Shoulder_basis_N24:1 ↔ DIN 934 - ersetzt durch DIN EN 24032/28673/28674 M4:12
- Passend:330 [Mate]: Shoulder_basis_N24:1 ↔ DIN 934 - ersetzt durch DIN EN 24032/28673/28674 M4:13
- Passend:331 [Mate]: Shoulder_basis_N24:1 ↔ Diszanzbolzen_M4x20:11
- Passend:332 [Mate]: Shoulder_basis_N24:1 ↔ Diszanzbolzen_M4x20:12
- Passend:333 [Mate]: Shoulder_basis_N24:1 ↔ Diszanzbolzen_M4x20:9
- Passend:334 [Mate]: Shoulder_basis_N24:1 ↔ Diszanzbolzen_M4x20:10
- Passend:335 [Mate]: Shoulder_basis_N24:1 ↔ Diszanzbolzen_M4x20:11
- Passend:336 [Mate]: Shoulder_basis_N24:1 ↔ Diszanzbolzen_M4x20:12
- Passend:337 [Mate]: Shoulder_basis_N24:1 ↔ Diszanzbolzen_M4x20:12
- Passend:338 [Mate]: Shoulder_basis_N24:1 ↔ Diszanzbolzen_M4x20:11
- Passend:339 [Mate]: Shoulder_basis_N24:1 ↔ Diszanzbolzen_M4x20:9
- Passend:340 [Mate]: Shoulder_basis_N24:1 ↔ Diszanzbolzen_M4x20:10
- Passend:341 [Mate]: Shoulder_basis_N24:1 ↔ Diszanzbolzen_M4x20:10
- Passend:342 [Mate]: Shoulder_basis_N24:1 ↔ Diszanzbolzen_M4x20:9
- Passend:344 [Mate]: Shoulder_basis_N24:1 ↔ DIN 912 - ersetzt durch DIN EN ISO 4762 M4 x 50:2
- Passend:345 [Mate]: Shoulder_basis_N24:1 ↔ DIN 912 - ersetzt durch DIN EN ISO 4762 M4 x 50:5
- Passend:346 [Mate]: Shoulder_basis_N24:1 ↔ DIN 912 - ersetzt durch DIN EN ISO 4762 M4 x 50:2
- Passend:347 [Mate]: Diszanzbolzen_M4x20:9 ↔ DIN 912 - ersetzt durch DIN EN ISO 4762 M4 x 50:3
- Passend:348 [Mate]: DIN 912 - ersetzt durch DIN EN ISO 4762 M4 x 50:3 ↔ DIN 912 - ersetzt durch DIN EN ISO 4762 M4 x 50:4
- Passend:349 [Mate]: Diszanzbolzen_M4x20:11 ↔ DIN 912 - ersetzt durch DIN EN ISO 4762 M4 x 60:17
- Passend:350 [Mate]: DIN 912 - ersetzt durch DIN EN ISO 4762 M4 x 60:16 ↔ DIN 912 - ersetzt durch DIN EN ISO 4762 M4 x 60:17
- Passend:351 [Mate]: Diszanzbolzen_M4x20:10 ↔ DIN 912 - ersetzt durch DIN EN ISO 4762 M4 x 60:19
- Passend:352 [Mate]: DIN 912 - ersetzt durch DIN EN ISO 4762 M4 x 60:18 ↔ DIN 912 - ersetzt durch DIN EN ISO 4762 M4 x 60:19
- Passend:353 [Mate]: Shoulder_basis_N24:1 ↔ DIN 912 - ersetzt durch DIN EN ISO 4762 M4 x 50:4
- Passend:354 [Mate]: Shoulder_basis_N24:1 ↔ DIN 912 - ersetzt durch DIN EN ISO 4762 M4 x 60:18
- Passend:355 [Mate]: Shoulder_basis_N24:1 ↔ DIN 912 - ersetzt durch DIN EN ISO 4762 M4 x 60:16
- Passend:356 [Mate]: Shoulder_basis_N24:1 ↔ DIN 912 - ersetzt durch DIN EN ISO 4762 M4 x 50:5
- Passend:357 [Mate]: Shoulder_basis_N24:1 ↔ DIN 912 - ersetzt durch DIN EN ISO 4762 M4 x 60:17
- Passend:358 [Mate]: Shoulder_basis_N24:1 ↔ DIN 912 - ersetzt durch DIN EN ISO 4762 M4 x 60:19
- Passend:359 [Mate]: Shoulder_basis_N24:1 ↔ DIN 912 - ersetzt durch DIN EN ISO 4762 M4 x 50:3
- Passend:360 [Mate]: Diszanzbolzen_M4x20:8 ↔ DIN 912 - ersetzt durch DIN EN ISO 4762 M4 x 70:25
- Passend:361 [Mate]: Diszanzbolzen_M4x20:4 ↔ DIN 912 - ersetzt durch DIN EN ISO 4762 M4 x 70:20
- Passend:362 [Mate]: Diszanzbolzen_M4x20:5 ↔ DIN 912 - ersetzt durch DIN EN ISO 4762 M4 x 70:21
- Passend:363 [Mate]: Diszanzbolzen_M4x20:6 ↔ DIN 912 - ersetzt durch DIN EN ISO 4762 M4 x 70:24
- Passend:364 [Mate]: Diszanzbolzen_M4x20:7 ↔ DIN 912 - ersetzt durch DIN EN ISO 4762 M4 x 70:22
- Passend:365 [Mate]: Diszanzbolzen_M4x20:3 ↔ DIN 912 - ersetzt durch DIN EN ISO 4762 M4 x 70:26
- Passend:366 [Mate]: Diszanzbolzen_M4x20:2 ↔ DIN 912 - ersetzt durch DIN EN ISO 4762 M4 x 70:27
- Fluchtend:44 [Flush]: DIN 912 - ersetzt durch DIN EN ISO 4762 M4 x 70:26 ↔ DIN 912 - ersetzt durch DIN EN ISO 4762 M4 x 70:27
- Fluchtend:45 [Flush]: DIN 912 - ersetzt durch DIN EN ISO 4762 M4 x 70:15 ↔ DIN 912 - ersetzt durch DIN EN ISO 4762 M4 x 70:27
- Fluchtend:46 [Flush]: DIN 912 - ersetzt durch DIN EN ISO 4762 M4 x 70:15 ↔ DIN 912 - ersetzt durch DIN EN ISO 4762 M4 x 70:25
- Fluchtend:47 [Flush]: DIN 912 - ersetzt durch DIN EN ISO 4762 M4 x 70:20 ↔ DIN 912 - ersetzt durch DIN EN ISO 4762 M4 x 70:21
- Fluchtend:48 [Flush]: DIN 912 - ersetzt durch DIN EN ISO 4762 M4 x 70:20 ↔ DIN 912 - ersetzt durch DIN EN ISO 4762 M4 x 70:25
- Fluchtend:49 [Flush]: DIN 912 - ersetzt durch DIN EN ISO 4762 M4 x 70:20 ↔ DIN 912 - ersetzt durch DIN EN ISO 4762 M4 x 70:24
- Fluchtend:50 [Flush]: DIN 912 - ersetzt durch DIN EN ISO 4762 M4 x 70:22 ↔ DIN 912 - ersetzt durch DIN EN ISO 4762 M4 x 70:24
- Passend:367 [Mate]: Shoulder_basis_N24:1 ↔ DIN 7991 M3x25:1
- Tangential:1: DIN 625 SKF SKF 61818:2 ↔ DIN 7991 M3x25:1
- Passend:368 [Mate]: DIN 934 - ersetzt durch DIN EN 24032/28673/28674 M3:1 ↔ DIN 7991 M3x25:1
- Passend:369 [Mate]: Shoulder_basis_N24:1 ↔ DIN 934 - ersetzt durch DIN EN 24032/28673/28674 M3:1
- Passend:370 [Mate]: Shoulder_basis_N24:1 ↔ DIN 934 - ersetzt durch DIN EN 24032/28673/28674 M3:1
- Passend:371 [Mate]: Shoulder_basis_N24:1 ↔ DIN 7991 M3x25:8
- Passend:373 [Mate]: DIN 7991 M3x25:8 ↔ DIN 934 - ersetzt durch DIN EN 24032/28673/28674 M3:8
- Passend:374 [Mate]: Shoulder_basis_N24:1 ↔ DIN 934 - ersetzt durch DIN EN 24032/28673/28674 M3:8
- Passend:375 [Mate]: Shoulder_basis_N24:1 ↔ DIN 934 - ersetzt durch DIN EN 24032/28673/28674 M3:8
- Tangential:2: DIN 625 SKF SKF 61818:1 ↔ DIN 7991 M3x25:8
